# Autodesk Inventor assembly: Trunk
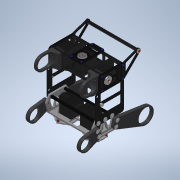
[picture p0: Inventor's stored thumbnail of the model, 180x180]
Saved by Autodesk Inventor 2022 (Build 260153000, 153)
## iProperties
Created: 2022-01-06
Part Number: Trunk
Document SubType Name: Assembly
Designer: Masato Kubotera
Mass: 836.462 g
Surface Area: 2738.45 cm^2
Volume: 519.507 cm^3
Density: 1.61011 g/cm^3
Author: Masato Kubotera
## Documents named in this file (27)
- C:\Users\MasatoKubotera\Documents\Inventor\SUSTAINA-OP\UpperBody\Trunk\Trunk.iam
- C:\Users\MasatoKubotera\Documents\Inventor\SUSTAINA-OP\ReadyMade\KONDO\B3M-SC-1170-A.ipt
- C:\Users\MasatoKubotera\Documents\Inventor\SUSTAINA-OP\UpperBody\Trunk\Trunk_chest_frame.ipt
- C:\Users\MasatoKubotera\Documents\Inventor\SUSTAINA-OP\ReadyMade\InsertNut\IRU-304S.ipt
- C:\Users\MasatoKubotera\Documents\Inventor\SUSTAINA-OP\UpperBody\Trunk\Trunk_neck_frame.ipt
- C:\Users\MasatoKubotera\Documents\Inventor\SUSTAINA-OP\ReadyMade\Screw\M2_6-15.ipt
- C:\Users\MasatoKubotera\Documents\Inventor\SUSTAINA-OP\ReadyMade\Screw\M3-6.ipt
- C:\Users\MasatoKubotera\Documents\Inventor\SUSTAINA-OP\ReadyMade\Screw\M3-8.ipt
- C:\Users\MasatoKubotera\Documents\Inventor\SUSTAINA-OP\UpperBody\Trunk\Trunk_shoulder_frame.ipt
- C:\Users\MasatoKubotera\Documents\Inventor\SUSTAINA-OP\UpperBody\Trunk\Trunk_upper_side_frame.ipt
- C:\Users\MasatoKubotera\Documents\Inventor\SUSTAINA-OP\ReadyMade\Screw\M3-10.ipt
- C:\Users\MasatoKubotera\Documents\Inventor\SUSTAINA-OP\UpperBody\Trunk\Trunk_shoulder_frame_MIR.ipt
- C:\Users\MasatoKubotera\Documents\Inventor\SUSTAINA-OP\ReadyMade\Washer\UUW-0312-10H.ipt
- C:\Users\MasatoKubotera\Documents\Inventor\SUSTAINA-OP\UpperBody\Trunk\Trunk_lower_side_frame.ipt
- C:\Users\MasatoKubotera\Documents\Inventor\SUSTAINA-OP\UpperBody\Trunk\Trunk_waisit_frame.ipt
- C:\Users\MasatoKubotera\Documents\Inventor\SUSTAINA-OP\UpperBody\Trunk\CrossRollerBearing\BearingUnit.iam
- C:\Users\MasatoKubotera\Documents\Inventor\SUSTAINA-OP\ReadyMade\Screw\SPNFL-BRN-M3-6.ipt
- C:\Users\MasatoKubotera\Documents\Inventor\SUSTAINA-OP\ReadyMade\Spacer\ABLSBF7-140-M3-N3.ipt
- C:\Users\MasatoKubotera\Documents\Inventor\SUSTAINA-OP\ReadyMade\Spacer\SLSBF7-157-M3-N3.ipt
- C:\Users\MasatoKubotera\Documents\Inventor\SUSTAINA-OP\ReadyMade\Spacer\BRU-309S.ipt
- C:\Users\MasatoKubotera\Documents\Inventor\SUSTAINA-OP\UpperBody\Trunk\Trunk_servo_bottom_frame.ipt
- C:\Users\MasatoKubotera\Documents\Inventor\SUSTAINA-OP\ReadyMade\KONDO\B3M-SC-1040-A_with_ClampHorn.iam
- C:\Users\MasatoKubotera\Documents\Inventor\SUSTAINA-OP\UpperBody\Trunk\FrontBumper.ipt
- C:\Users\MasatoKubotera\Documents\Inventor\SUSTAINA-OP\UpperBody\Trunk\RearBumper.ipt
- C:\Users\MasatoKubotera\Documents\Inventor\SUSTAINA-OP\UpperBody\Trunk\ChestBumper.ipt
- C:\Users\MasatoKubotera\Documents\Inventor\SUSTAINA-OP\UpperBody\Trunk\Trunk_chest_frame_cover_sheet.ipt
- C:\Users\MasatoKubotera\Documents\Inventor\SUSTAINA-OP\UpperBody\Trunk\Handle_ShrinkTube.ipt
## Components (105 placed, 27 different names)
1. BearingUnit:1 [sub-assembly] — 挿入:83, 挿入:84
2. BearingUnit:2 [sub-assembly] — 挿入:85, 挿入:86
3. Handle_ShrinkTube:1 — フラッシュ:11, フラッシュ:12, メイト:5
4. Trunk_shoulder_frame:1 — 挿入:33, 挿入:34, 挿入:35, 挿入:36, 挿入:37, 挿入:39, 挿入:38, 挿入:40, 挿入:139, 挿入:206, 挿入:207, メイト:5
5. Trunk_shoulder_frame_MIR:1 — 挿入:56, 挿入:57, 挿入:58, 挿入:59, 挿入:65, 挿入:66, 挿入:67, 挿入:68, 角度:5, 挿入:141, 挿入:208, 挿入:209
6. Trunk_upper_side_frame:1 — 挿入:29, 挿入:30, 挿入:31, 挿入:32, 挿入:33, 挿入:34, 挿入:35, 挿入:36, 挿入:5, 挿入:119, 挿入:195, 挿入:196, メイト:4, 挿入:226, 挿入:227, 挿入:228
7. Trunk_upper_side_frame:2 — 挿入:52, 挿入:53, 挿入:54, 挿入:55, 挿入:56, 挿入:57, 挿入:58, 挿入:59, 挿入:120, メイト:3, 挿入:229, 挿入:230, 挿入:231
8. Trunk_neck_frame:1 — 挿入:18, 挿入:20, 挿入:25, 挿入:26, 挿入:27, 挿入:28, 挿入:204, 挿入:205
9. Trunk_chest_frame:1 — 挿入:2, 挿入:3, 挿入:4, 挿入:6, 挿入:131
10. Trunk_chest_frame:2 — 挿入:7, 挿入:9, 挿入:10, 挿入:11, 挿入:12, 挿入:8, メイト:1, メイト:2, フラッシュ:5, フラッシュ:6, フラッシュ:7, フラッシュ:8, フラッシュ:9, フラッシュ:10
11. Trunk_waisit_frame:1 — フラッシュ:2, フラッシュ:3, フラッシュ:4, 挿入:83, 挿入:84, 挿入:85, 挿入:86, 挿入:87, 挿入:88, 挿入:89, 挿入:90, 挿入:91, 挿入:92, 挿入:93, 挿入:94, 挿入:121, 挿入:122, 挿入:123, 挿入:124, 挿入:143, 挿入:144, 挿入:177, 挿入:178
12. Trunk_lower_side_frame:1 — 挿入:177, 挿入:178, 角度:6, 角度:7, 挿入:179, 挿入:180, 挿入:195, 挿入:196, 挿入:214, 挿入:215, 挿入:216, 挿入:217
13. Trunk_lower_side_frame:2 — 挿入:143, 挿入:144, 挿入:210, 挿入:211, 挿入:212, 挿入:213
14. Trunk_servo_bottom_frame:1
15. Trunk_servo_bottom_frame:2
16. Trunk_servo_bottom_frame:3
17. Trunk_chest_frame_cover_sheet:1 — フラッシュ:7, フラッシュ:8, フラッシュ:9, フラッシュ:10
18. ChestBumper:2 — メイト:2, メイト:4, フラッシュ:6
19. ChestBumper:1 — メイト:1, メイト:3, フラッシュ:5
20. RearBumper:2 — 挿入:224, 挿入:225
21. FrontBumper:2 — 挿入:222, 挿入:223
22. RearBumper:1 — 挿入:220, 挿入:221
23. FrontBumper:1 — 挿入:218, 挿入:219
24. BRU-309S:1 — 挿入:161, 挿入:214
25. BRU-309S:2 — 挿入:162, 挿入:215
26. BRU-309S:3 — 挿入:163, 挿入:216
27. BRU-309S:4 — 挿入:164, 挿入:217
28. BRU-309S:5 — 挿入:165, 挿入:210
29. BRU-309S:6 — 挿入:166, 挿入:211
30. BRU-309S:7 — 挿入:167, 挿入:212
31. BRU-309S:8 — 挿入:168, 挿入:213
32. UUW-0312-10H:1 — 挿入:75, 挿入:140
33. UUW-0312-10H:2 — 挿入:76, 挿入:142
34. UUW-0312-10H:11 — 挿入:161, 挿入:169, 挿入:218
35. UUW-0312-10H:12 — 挿入:162, 挿入:170, 挿入:219
36. UUW-0312-10H:13 — 挿入:163, 挿入:171, 挿入:220
37. UUW-0312-10H:14 — 挿入:164, 挿入:172, 挿入:221
38. UUW-0312-10H:15 — 挿入:165, 挿入:173, 挿入:224
39. UUW-0312-10H:16 — 挿入:166, 挿入:174, 挿入:225
40. UUW-0312-10H:17 — 挿入:167, 挿入:175, 挿入:222
41. UUW-0312-10H:18 — 挿入:168, 挿入:176, 挿入:223
42. UUW-0312-10H:19 — 挿入:189, 挿入:226
43. UUW-0312-10H:20 — 挿入:193, 挿入:227
44. UUW-0312-10H:21 — 挿入:190, 挿入:228
45. UUW-0312-10H:22 — 挿入:191, 挿入:229
46. UUW-0312-10H:23 — 挿入:194, 挿入:230
47. UUW-0312-10H:24 — 挿入:192, 挿入:231
48. SLSBF7-157-M3-N3:1 — 角度:5, 挿入:139, 挿入:140, 挿入:141, 挿入:142, フラッシュ:11, フラッシュ:12
49. ABLSBF7-140-M3-N3:1 — 角度:6, 挿入:179
50. ABLSBF7-140-M3-N3:2 — 角度:7, 挿入:180
51. B3M-SC-1170-A:2 — 挿入:89, 挿入:90
52. B3M-SC-1170-A:1 — 挿入:87, 挿入:88
53. B3M-SC-1040-A_with_ClampHorn:1 [sub-assembly] — 挿入:204, 挿入:205
54. B3M-SC-1040-A_with_ClampHorn:2 [sub-assembly] — 挿入:206, 挿入:207
55. B3M-SC-1040-A_with_ClampHorn:3 [sub-assembly] — 挿入:208, 挿入:209
56. IRU-304S:12 — 挿入:12, 挿入:53
57. IRU-304S:11 — 挿入:11, 挿入:52
58. IRU-304S:10 — 挿入:10, 挿入:30
59. IRU-304S:9 — 挿入:9, 挿入:29
60. IRU-304S:8 — 挿入:8
61. IRU-304S:7 — 挿入:7, 挿入:18
62. IRU-304S:6 — 挿入:6, 挿入:32
63. IRU-304S:5 — 挿入:5, 挿入:31
64. IRU-304S:4 — 挿入:4, 挿入:55
65. IRU-304S:3 — 挿入:3, 挿入:54
66. IRU-304S:2 — 挿入:2, 挿入:20
67. IRU-304SW:1 — 挿入:131
68. M3-6:9 — 挿入:169
69. M3-6:10 — 挿入:170
70. M3-6:11 — 挿入:171
71. M3-6:12 — 挿入:172
72. M3-6:13 — 挿入:173
73. M3-6:14 — 挿入:174
74. M3-6:15 — 挿入:176
75. M3-6:16 — 挿入:175
76. M3-10:17 — 挿入:189
77. M3-10:18 — 挿入:190
78. M3-10:19 — 挿入:191
79. M3-10:20 — 挿入:192
80. M3-8:7 — 挿入:193
81. M3-8:8 — 挿入:194
82. M3-10:13 — 挿入:121
83. M3-10:14 — 挿入:122
84. M3-10:15 — 挿入:123
85. M3-10:16 — 挿入:124
86. SPNFL-BRN-M3-6:1 — 挿入:119
87. SPNFL-BRN-M3-6:2 — 挿入:120
88. M3-8:2 — 挿入:28
89. M3-8:1 — 挿入:27
90. M3-6:2 — 挿入:26
91. M3-6:1 — 挿入:25
92. M3-8:4 — 挿入:38
93. M3-8:3 — 挿入:37
94. M3-10:4 — 挿入:40
95. M3-10:3 — 挿入:39
96. M3-10:6 — 挿入:68
97. M3-10:5 — 挿入:67
98. M3-8:6 — 挿入:66
99. M3-8:5 — 挿入:65
100. M3-6:4 — 挿入:76
101. M3-6:3 — 挿入:75
102. M2_6-15:16 — 挿入:94
103. M2_6-15:15 — 挿入:93
104. M2_6-15:14 — 挿入:92
105. M2_6-15:13 — 挿入:91
## Relationships (143: Insert 124, Flush 11, Mate 5, Angle 3)
- 挿入:2 [Insert]: Trunk_chest_frame:1 ↔ IRU-304S:2
- 挿入:3 [Insert]: Trunk_chest_frame:1 ↔ IRU-304S:3
- 挿入:4 [Insert]: Trunk_chest_frame:1 ↔ IRU-304S:4
- 挿入:5 [Insert]: Trunk_upper_side_frame:1 ↔ IRU-304S:5
- 挿入:6 [Insert]: Trunk_chest_frame:1 ↔ IRU-304S:6
- 挿入:7 [Insert]: Trunk_chest_frame:2 ↔ IRU-304S:7
- 挿入:8 [Insert]: Trunk_chest_frame:2 ↔ IRU-304S:8
- 挿入:9 [Insert]: Trunk_chest_frame:2 ↔ IRU-304S:9
- 挿入:10 [Insert]: Trunk_chest_frame:2 ↔ IRU-304S:10
- 挿入:11 [Insert]: Trunk_chest_frame:2 ↔ IRU-304S:11
- 挿入:12 [Insert]: Trunk_chest_frame:2 ↔ IRU-304S:12
- 挿入:18 [Insert]: Trunk_neck_frame:1 ↔ IRU-304S:7
- 挿入:20 [Insert]: Trunk_neck_frame:1 ↔ IRU-304S:2
- 挿入:25 [Insert]: Trunk_neck_frame:1 ↔ M3-6:1
- 挿入:26 [Insert]: Trunk_neck_frame:1 ↔ M3-6:2
- 挿入:27 [Insert]: Trunk_neck_frame:1 ↔ M3-8:1
- 挿入:28 [Insert]: Trunk_neck_frame:1 ↔ M3-8:2
- 挿入:29 [Insert]: Trunk_upper_side_frame:1 ↔ IRU-304S:9
- 挿入:30 [Insert]: Trunk_upper_side_frame:1 ↔ IRU-304S:10
- 挿入:31 [Insert]: Trunk_upper_side_frame:1 ↔ IRU-304S:5
- 挿入:32 [Insert]: Trunk_upper_side_frame:1 ↔ IRU-304S:6
- 挿入:33 [Insert]: Trunk_shoulder_frame:1 ↔ Trunk_upper_side_frame:1
- 挿入:34 [Insert]: Trunk_shoulder_frame:1 ↔ Trunk_upper_side_frame:1
- 挿入:35 [Insert]: Trunk_shoulder_frame:1 ↔ Trunk_upper_side_frame:1
- 挿入:36 [Insert]: Trunk_shoulder_frame:1 ↔ Trunk_upper_side_frame:1
- 挿入:37 [Insert]: Trunk_shoulder_frame:1 ↔ M3-8:3
- 挿入:39 [Insert]: Trunk_shoulder_frame:1 ↔ M3-10:3
- 挿入:38 [Insert]: Trunk_shoulder_frame:1 ↔ M3-8:4
- 挿入:40 [Insert]: Trunk_shoulder_frame:1 ↔ M3-10:4
- 挿入:52 [Insert]: Trunk_upper_side_frame:2 ↔ IRU-304S:11
- 挿入:53 [Insert]: Trunk_upper_side_frame:2 ↔ IRU-304S:12
- 挿入:54 [Insert]: Trunk_upper_side_frame:2 ↔ IRU-304S:3
- 挿入:55 [Insert]: Trunk_upper_side_frame:2 ↔ IRU-304S:4
- 挿入:56 [Insert]: Trunk_shoulder_frame_MIR:1 ↔ Trunk_upper_side_frame:2
- 挿入:57 [Insert]: Trunk_shoulder_frame_MIR:1 ↔ Trunk_upper_side_frame:2
- 挿入:58 [Insert]: Trunk_shoulder_frame_MIR:1 ↔ Trunk_upper_side_frame:2
- 挿入:59 [Insert]: Trunk_shoulder_frame_MIR:1 ↔ Trunk_upper_side_frame:2
- 挿入:65 [Insert]: Trunk_shoulder_frame_MIR:1 ↔ M3-8:5
- 挿入:66 [Insert]: Trunk_shoulder_frame_MIR:1 ↔ M3-8:6
- 挿入:67 [Insert]: Trunk_shoulder_frame_MIR:1 ↔ M3-10:5
- 挿入:68 [Insert]: Trunk_shoulder_frame_MIR:1 ↔ M3-10:6
- 挿入:75 [Insert]: UUW-0312-10H:1 ↔ M3-6:3
- 挿入:76 [Insert]: UUW-0312-10H:2 ↔ M3-6:4
- フラッシュ:2 [Flush]: Trunk_waisit_frame:1
- フラッシュ:3 [Flush]: Trunk_waisit_frame:1
- フラッシュ:4 [Flush]: Trunk_waisit_frame:1
- 挿入:83 [Insert]: BearingUnit:1 ↔ Trunk_waisit_frame:1
- 挿入:84 [Insert]: BearingUnit:1 ↔ Trunk_waisit_frame:1
- 挿入:85 [Insert]: BearingUnit:2 ↔ Trunk_waisit_frame:1
- 挿入:86 [Insert]: BearingUnit:2 ↔ Trunk_waisit_frame:1
- 挿入:87 [Insert]: Trunk_waisit_frame:1 ↔ B3M-SC-1170-A:1
- 挿入:88 [Insert]: Trunk_waisit_frame:1 ↔ B3M-SC-1170-A:1
- 挿入:89 [Insert]: Trunk_waisit_frame:1 ↔ B3M-SC-1170-A:2
- 挿入:90 [Insert]: Trunk_waisit_frame:1 ↔ B3M-SC-1170-A:2
- 挿入:91 [Insert]: Trunk_waisit_frame:1 ↔ M2_6-15:13
- 挿入:92 [Insert]: Trunk_waisit_frame:1 ↔ M2_6-15:14
- 挿入:93 [Insert]: Trunk_waisit_frame:1 ↔ M2_6-15:15
- 挿入:94 [Insert]: Trunk_waisit_frame:1 ↔ M2_6-15:16
- 挿入:119 [Insert]: Trunk_upper_side_frame:1 ↔ SPNFL-BRN-M3-6:1
- 挿入:120 [Insert]: Trunk_upper_side_frame:2 ↔ SPNFL-BRN-M3-6:2
- 挿入:121 [Insert]: Trunk_waisit_frame:1 ↔ M3-10:13
- 挿入:122 [Insert]: Trunk_waisit_frame:1 ↔ M3-10:14
- 挿入:123 [Insert]: Trunk_waisit_frame:1 ↔ M3-10:15
- 挿入:124 [Insert]: Trunk_waisit_frame:1 ↔ M3-10:16
- 挿入:131 [Insert]: Trunk_chest_frame:1 ↔ IRU-304SW:1
- 角度:5 [Angle] (0 deg): Trunk_shoulder_frame_MIR:1 ↔ SLSBF7-157-M3-N3:1
- 挿入:139 [Insert]: Trunk_shoulder_frame:1 ↔ SLSBF7-157-M3-N3:1
- 挿入:140 [Insert]: UUW-0312-10H:1 ↔ SLSBF7-157-M3-N3:1
- 挿入:141 [Insert]: Trunk_shoulder_frame_MIR:1 ↔ SLSBF7-157-M3-N3:1
- 挿入:142 [Insert]: UUW-0312-10H:2 ↔ SLSBF7-157-M3-N3:1
- 挿入:143 [Insert]: Trunk_waisit_frame:1 ↔ Trunk_lower_side_frame:2
- 挿入:144 [Insert]: Trunk_waisit_frame:1 ↔ Trunk_lower_side_frame:2
- 挿入:161 [Insert]: BRU-309S:1 ↔ UUW-0312-10H:11
- 挿入:162 [Insert]: BRU-309S:2 ↔ UUW-0312-10H:12
- 挿入:163 [Insert]: BRU-309S:3 ↔ UUW-0312-10H:13
- 挿入:164 [Insert]: BRU-309S:4 ↔ UUW-0312-10H:14
- 挿入:165 [Insert]: BRU-309S:5 ↔ UUW-0312-10H:15
- 挿入:166 [Insert]: BRU-309S:6 ↔ UUW-0312-10H:16
- 挿入:167 [Insert]: BRU-309S:7 ↔ UUW-0312-10H:17
- 挿入:168 [Insert]: BRU-309S:8 ↔ UUW-0312-10H:18
- 挿入:169 [Insert]: UUW-0312-10H:11 ↔ M3-6:9
- 挿入:170 [Insert]: UUW-0312-10H:12 ↔ M3-6:10
- 挿入:171 [Insert]: UUW-0312-10H:13 ↔ M3-6:11
- 挿入:172 [Insert]: UUW-0312-10H:14 ↔ M3-6:12
- 挿入:173 [Insert]: UUW-0312-10H:15 ↔ M3-6:13
- 挿入:174 [Insert]: UUW-0312-10H:16 ↔ M3-6:14
- 挿入:175 [Insert]: UUW-0312-10H:17 ↔ M3-6:16
- 挿入:176 [Insert]: UUW-0312-10H:18 ↔ M3-6:15
- 挿入:177 [Insert]: Trunk_waisit_frame:1 ↔ Trunk_lower_side_frame:1
- 挿入:178 [Insert]: Trunk_waisit_frame:1 ↔ Trunk_lower_side_frame:1
- 角度:6 [Angle] (0 deg): Trunk_lower_side_frame:1 ↔ ABLSBF7-140-M3-N3:1
- 角度:7 [Angle] (0 deg): Trunk_lower_side_frame:1 ↔ ABLSBF7-140-M3-N3:2
- 挿入:179 [Insert]: Trunk_lower_side_frame:1 ↔ ABLSBF7-140-M3-N3:1
- 挿入:180 [Insert]: Trunk_lower_side_frame:1 ↔ ABLSBF7-140-M3-N3:2
- 挿入:189 [Insert]: UUW-0312-10H:19 ↔ M3-10:17
- 挿入:190 [Insert]: UUW-0312-10H:21 ↔ M3-10:18
- 挿入:191 [Insert]: UUW-0312-10H:22 ↔ M3-10:19
- 挿入:192 [Insert]: UUW-0312-10H:24 ↔ M3-10:20
- 挿入:193 [Insert]: UUW-0312-10H:20 ↔ M3-8:7
- 挿入:194 [Insert]: UUW-0312-10H:23 ↔ M3-8:8
- 挿入:195 [Insert]: Trunk_upper_side_frame:1 ↔ Trunk_lower_side_frame:1
- 挿入:196 [Insert]: Trunk_upper_side_frame:1 ↔ Trunk_lower_side_frame:1
- 挿入:204 [Insert]: Trunk_neck_frame:1 ↔ B3M-SC-1040-A_with_ClampHorn:1
- 挿入:205 [Insert]: Trunk_neck_frame:1 ↔ B3M-SC-1040-A_with_ClampHorn:1
- 挿入:206 [Insert]: Trunk_shoulder_frame:1 ↔ B3M-SC-1040-A_with_ClampHorn:2
- 挿入:207 [Insert]: Trunk_shoulder_frame:1 ↔ B3M-SC-1040-A_with_ClampHorn:2
- 挿入:208 [Insert]: Trunk_shoulder_frame_MIR:1 ↔ B3M-SC-1040-A_with_ClampHorn:3
- 挿入:209 [Insert]: Trunk_shoulder_frame_MIR:1 ↔ B3M-SC-1040-A_with_ClampHorn:3
- 挿入:210 [Insert]: Trunk_lower_side_frame:2 ↔ BRU-309S:5
- 挿入:211 [Insert]: Trunk_lower_side_frame:2 ↔ BRU-309S:6
- 挿入:212 [Insert]: Trunk_lower_side_frame:2 ↔ BRU-309S:7
- 挿入:213 [Insert]: Trunk_lower_side_frame:2 ↔ BRU-309S:8
- 挿入:214 [Insert]: Trunk_lower_side_frame:1 ↔ BRU-309S:1
- 挿入:215 [Insert]: Trunk_lower_side_frame:1 ↔ BRU-309S:2
- 挿入:216 [Insert]: Trunk_lower_side_frame:1 ↔ BRU-309S:3
- 挿入:217 [Insert]: Trunk_lower_side_frame:1 ↔ BRU-309S:4
- 挿入:218 [Insert]: FrontBumper:1 ↔ UUW-0312-10H:11
- 挿入:219 [Insert]: FrontBumper:1 ↔ UUW-0312-10H:12
- 挿入:220 [Insert]: RearBumper:1 ↔ UUW-0312-10H:13
- 挿入:221 [Insert]: RearBumper:1 ↔ UUW-0312-10H:14
- 挿入:222 [Insert]: FrontBumper:2 ↔ UUW-0312-10H:17
- 挿入:223 [Insert]: FrontBumper:2 ↔ UUW-0312-10H:18
- 挿入:224 [Insert]: RearBumper:2 ↔ UUW-0312-10H:15
- 挿入:225 [Insert]: RearBumper:2 ↔ UUW-0312-10H:16
- メイト:1 [Mate]: Trunk_chest_frame:2 ↔ ChestBumper:1
- メイト:2 [Mate]: Trunk_chest_frame:2 ↔ ChestBumper:2
- メイト:3 [Mate]: Trunk_upper_side_frame:2 ↔ ChestBumper:1
- メイト:4 [Mate]: Trunk_upper_side_frame:1 ↔ ChestBumper:2
- フラッシュ:5 [Flush]: Trunk_chest_frame:2 ↔ ChestBumper:1
- フラッシュ:6 [Flush]: Trunk_chest_frame:2 ↔ ChestBumper:2
- フラッシュ:7 [Flush]: Trunk_chest_frame:2 ↔ Trunk_chest_frame_cover_sheet:1
- フラッシュ:8 [Flush]: Trunk_chest_frame:2 ↔ Trunk_chest_frame_cover_sheet:1
- フラッシュ:9 [Flush]: Trunk_chest_frame:2 ↔ Trunk_chest_frame_cover_sheet:1
- フラッシュ:10 [Flush]: Trunk_chest_frame:2 ↔ Trunk_chest_frame_cover_sheet:1
- 挿入:226 [Insert]: Trunk_upper_side_frame:1 ↔ UUW-0312-10H:19
- 挿入:227 [Insert]: Trunk_upper_side_frame:1 ↔ UUW-0312-10H:20
- 挿入:228 [Insert]: Trunk_upper_side_frame:1 ↔ UUW-0312-10H:21
- 挿入:229 [Insert]: Trunk_upper_side_frame:2 ↔ UUW-0312-10H:22
- 挿入:230 [Insert]: Trunk_upper_side_frame:2 ↔ UUW-0312-10H:23
- 挿入:231 [Insert]: Trunk_upper_side_frame:2 ↔ UUW-0312-10H:24
- フラッシュ:11 [Flush]: Handle_ShrinkTube:1 ↔ SLSBF7-157-M3-N3:1
- フラッシュ:12 [Flush]: Handle_ShrinkTube:1 ↔ SLSBF7-157-M3-N3:1
- メイト:5 [Mate]: Handle_ShrinkTube:1 ↔ Trunk_shoulder_frame:1
